# Autodesk Inventor assembly: final_assembly_2017_SuperUltraLow
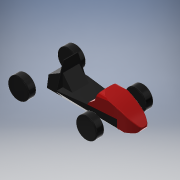
[picture p0: Inventor's stored thumbnail of the model, 180x180]
Saved by Autodesk Inventor 2018.1 (Build 221171000, 171)
## iProperties
Created: 2017-10-06
Part Number: final_assembly_2017_SuperUltraLow
Material: 一般
Document SubType Name: Assembly
Designer: kuwano
Sending System: Autodesk Inventor 2018
Preprocessor: ST-DEVELOPER v16.13
Title: D:\kuwano\Documents\Inventor\KITformula\CFD_KS-14\KS-14\stp\final_assembly_2017_SuperUltraLow.stp
Author: kuwano
## Documents named in this file (5)
- D:\kuwano\Documents\Inventor\KITformula\KS-15\KS-14_SULow\KS-14_SULow.iam
- D:\kuwano\Documents\Inventor\KITformula\KS-15\KS-14_SULow\parts\kaul_reretouch.ipt
- D:\kuwano\Documents\Inventor\KITformula\KS-15\KS-14_SULow\parts\newbody.ipt
- D:\kuwano\Documents\Inventor\KITformula\KS-15\KS-14_SULow\parts\tire_low.ipt
- D:\kuwano\Documents\Inventor\KITformula\KS-15\KS-14_SULow\parts\tire_low_MIR.ipt
## Components (6 placed, 4 different names)
1. kaul_retouch:1 — メイト:1, メイト:2, メイト:3
2. newbody:1 — フラッシュ:4, メイト:1, メイト:2, メイト:3
3. tire_low:1
4. tire_low:2
5. tire_low_MIR:1
6. tire_low_MIR:2
## Relationships (4: Mate 3, Flush 1)
- フラッシュ:4 [Flush]: newbody:1
- メイト:1 [Mate]: kaul_retouch:1 ↔ newbody:1
- メイト:2 [Mate]: kaul_retouch:1 ↔ newbody:1
- メイト:3 [Mate]: kaul_retouch:1 ↔ newbody:1
